# Autodesk Inventor assembly: Wheel & Motor
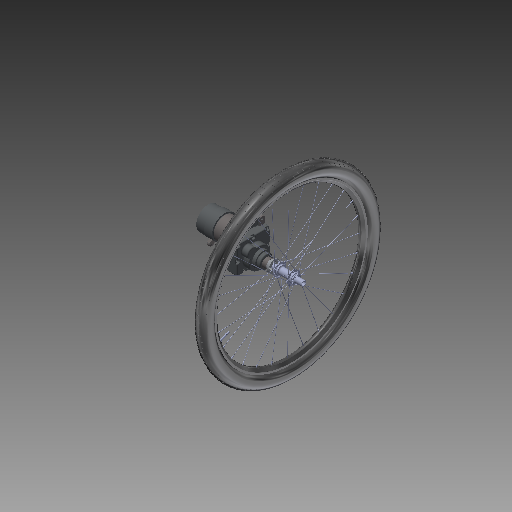
[picture p0: Inventor's stored thumbnail of the model, 512x512]
Saved by Autodesk Inventor 2017 SP1 (Build 210196100, 196)
## iProperties
Created: 2016-04-02
Part Number: Wheel & Motor
Document SubType Name: Assembly
Designer: hwasserb
Author: hwasserb
## Documents named in this file (4)
- C:\Users\Haden\Desktop\Charlie-CAD-Model\Robot Model\Motor\Motor and Tire.iam
- C:\Users\Haden\Desktop\Charlie-CAD-Model\Robot Model\Motor\NPC-T64 Motor.ipt
- C:\Users\Haden\Desktop\Charlie-CAD-Model\Robot Model\Motor\WHEEL_ADAPTER.ipt
- C:\Users\Haden\Desktop\Charlie-CAD-Model\Robot Model\Motor\Bike Wheel.ipt
## Components (3 placed, 3 different names)
1. NPC-T64 Motor:1 — Insert:1, Insert:2, Insert:3, Insert:4
2. WHEEL_ADAPTER:1 — Insert:1, Insert:2, Insert:3, Insert:4, Mate:1, Mate:2
3. Bike Wheel:1 — Mate:1, Mate:2
## Relationships (6: Insert 4, Mate 2)
- Insert:1: NPC-T64 Motor:1 ↔ WHEEL_ADAPTER:1
- Insert:2: NPC-T64 Motor:1 ↔ WHEEL_ADAPTER:1
- Insert:3: NPC-T64 Motor:1 ↔ WHEEL_ADAPTER:1
- Insert:4: NPC-T64 Motor:1 ↔ WHEEL_ADAPTER:1
- Mate:1: WHEEL_ADAPTER:1 ↔ Bike Wheel:1
- Mate:2 (-12.7 mm): WHEEL_ADAPTER:1 ↔ Bike Wheel:1
